# Autodesk Inventor assembly: Ensamblaje5
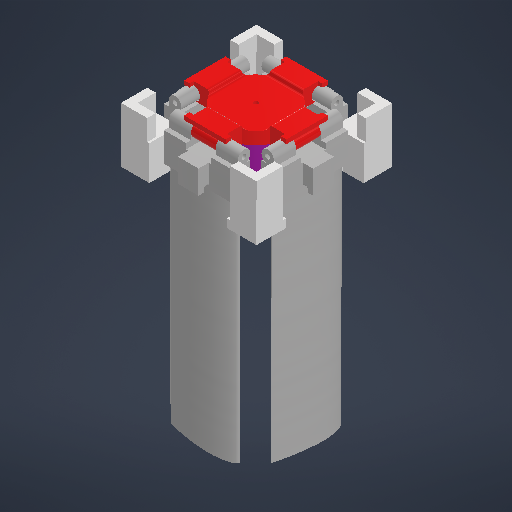
[picture p0: Inventor's stored thumbnail of the model, 512x512]
Saved by Autodesk Inventor 2026.1 (Build 301233000, 233)
## iProperties
Created: 2025-11-12
Part Number: Ensamblaje5
Document SubType Name: Assembly
Designer: usuario
Author: usuario
## Documents named in this file (5)
- C:\Users\usuario\Documents\vickh_Cansat\Cansat_Huitzilin\3D\NuevoDiseno\Ensamblaje5.iam
- C:\Users\usuario\Documents\vickh_Cansat\Cansat_Huitzilin\3D\NuevoDiseno\SujeccionHelices.ipt
- C:\Users\usuario\Documents\vickh_Cansat\Cansat_Huitzilin\3D\NuevoDiseno\SistemLiberacion1.ipt
- C:\Users\usuario\Documents\vickh_Cansat\Cansat_Huitzilin\3D\ViejoDiseno\Pieza9.ipt
- C:\Users\usuario\Documents\vickh_Cansat\Cansat_Huitzilin\3D\NuevoDiseno\SistemaLiberacion2.2.ipt
## Components (7 placed, 4 different names)
1. SujeccionHelices:1 — Cilíndrica:1, Nivelación:1, De rotación:1, De rotación:2, De rotación:3, De rotación:4
2. SistemLiberacion1:1 — Cilíndrica:1
3. Pieza9:1 — De rotación:1
4. Pieza9:2 — De rotación:3
5. Pieza9:3 — De rotación:4
6. Pieza9:4 — De rotación:2
7. SistemaLiberacion2.2:1 — Nivelación:1
## Relationships (6: RevoluteJoint 4, CylindricalJoint 1, Flush 1)
- Cilíndrica:1 [CylindricalJoint]: SujeccionHelices:1 ↔ SistemLiberacion1:1
- Nivelación:1 [Flush]: SujeccionHelices:1 ↔ SistemaLiberacion2.2:1
- De rotación:1 [RevoluteJoint]: SujeccionHelices:1 ↔ Pieza9:1
- De rotación:2 [RevoluteJoint]: SujeccionHelices:1 ↔ Pieza9:4
- De rotación:3 [RevoluteJoint]: SujeccionHelices:1 ↔ Pieza9:2
- De rotación:4 [RevoluteJoint]: SujeccionHelices:1 ↔ Pieza9:3
